# Autodesk Inventor assembly: RECOMPENSA
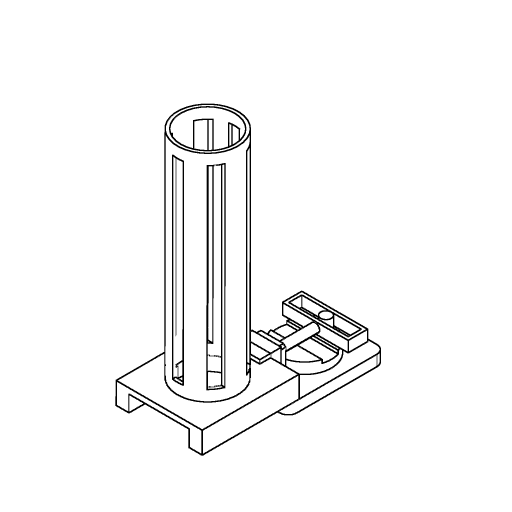
[picture p0: Inventor's stored thumbnail of the model, 512x512]
Saved by Autodesk Inventor 2024 (Build 280153000, 153)
## iProperties
Created: 2024-06-30
Part Number: RECOMPENSA
Document SubType Name: Assembly
Designer: Jhuliams
Author: Jhuliams
## Documents named in this file (7)
- C:\Users\Jhuliams\Documents\GitHub\RECICLADOR_MODELO_3D\MECANISMO DE RECOMPENSA\RECOMPENSA.iam
- C:\Users\Jhuliams\Documents\GitHub\RECICLADOR_MODELO_3D\MECANISMO DE RECOMPENSA\BASE DE YUGO ESCOCES.ipt
- C:\Users\Jhuliams\Documents\GitHub\RECICLADOR_MODELO_3D\MECANISMO DE RECOMPENSA\GUIA GIRATORIA.ipt
- C:\Users\Jhuliams\Documents\GitHub\RECICLADOR_MODELO_3D\MECANISMO DE RECOMPENSA\YUGO.ipt
- C:\Users\Jhuliams\Documents\GitHub\RECICLADOR_MODELO_3D\MECANISMO DE RECOMPENSA\RODAMIENTO LINEAL.ipt
- C:\Users\Jhuliams\Documents\GitHub\RECICLADOR_MODELO_3D\MECANISMO DE RECOMPENSA\PIN.ipt
- C:\Users\Jhuliams\Documents\GitHub\RECICLADOR_MODELO_3D\MECANISMO DE RECOMPENSA\TUBO CONTENEDOR.ipt
## Components (6 placed, 6 different names)
1. BASE DE YUGO ESCOCES:1 — Mate:1, Mate:5, Mate:7, Flush:2, Mate:11
2. GUIA GIRATORIA:1 — Mate:1, Mate:8, Mate:9
3. RODAMIENTO LINEAL:1 — Mate:5, Mate:6, Mate:7, Flush:2, Mate:10
4. YUGO:1 — Mate:6, Mate:8, Flush:3, Tangent:1
5. PIN:1 — Mate:9, Flush:3, Tangent:1
6. TUBO CONTENEDOR:1 — Mate:10, Mate:11
## Relationships (11: Mate 8, Flush 2, Tangent 1)
- Mate:1: BASE DE YUGO ESCOCES:1 ↔ GUIA GIRATORIA:1
- Mate:5: BASE DE YUGO ESCOCES:1 ↔ RODAMIENTO LINEAL:1
- Mate:6: RODAMIENTO LINEAL:1 ↔ YUGO:1
- Mate:7: BASE DE YUGO ESCOCES:1 ↔ RODAMIENTO LINEAL:1
- Flush:2 (1 mm): BASE DE YUGO ESCOCES:1 ↔ RODAMIENTO LINEAL:1
- Mate:8: GUIA GIRATORIA:1 ↔ YUGO:1
- Mate:9: GUIA GIRATORIA:1 ↔ PIN:1
- Flush:3: YUGO:1 ↔ PIN:1
- Tangent:1: YUGO:1 ↔ PIN:1
- Mate:10: RODAMIENTO LINEAL:1 ↔ TUBO CONTENEDOR:1
- Mate:11: BASE DE YUGO ESCOCES:1 ↔ TUBO CONTENEDOR:1
